# Autodesk Inventor assembly: Робот
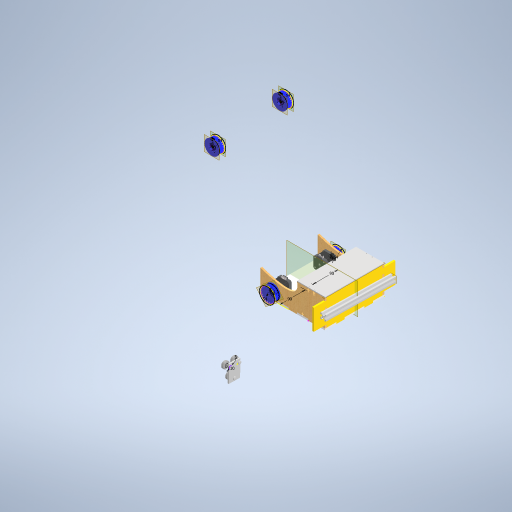
[picture p0: Inventor's stored thumbnail of the model, 512x512]
Saved by Autodesk Inventor 2024.2 (Build 282272000, 272)
## iProperties
Created: 2026-01-27
Part Number: Робот
Document SubType Name: Assembly
Designer: Service
d4: 0,000 мм
Author: Service
## Documents named in this file (9)
- C:\Users\Service\Documents\Artist-v2\3D\Робот.iam
- C:\Users\Service\Documents\Artist-v2\3D\Низ робота.ipt
- C:\Users\Service\Documents\Artist-v2\3D\бок.ipt
- C:\Users\Service\Documents\Artist-v2\3D\перед.ipt
- C:\Users\Service\Documents\Artist-v2\3D\в_профиль 2020.ipt
- C:\Users\Service\Documents\Artist-v2\3D\NEMA17 42-40.ipt
- C:\Users\Service\Documents\Artist-v2\3D\Шестерня.ipt
- C:\Users\Service\Documents\крышка.ipt
- C:\Users\Service\Documents\Artist-v2\3D\каретка.iam
## Components (13 placed, 8 different names)
1. Низ робота:1 — Заподлицо:1, Совмещение:1, Заподлицо:2, Симметрия:1, Совмещение:2, Заподлицо:3, Заподлицо:4, Совмещение:3, Заподлицо:5, Совмещение:12
2. бок:1 — Заподлицо:1, Совмещение:1, Заподлицо:2, Симметрия:1, Совмещение:4, Совмещение:5, Совмещение:13
3. бок:2 — Совмещение:2, Заподлицо:3, Заподлицо:4, Совмещение:6, Совмещение:7, Совмещение:8, Совмещение:10, Заподлицо:6
4. перед:1 — Совмещение:3, Заподлицо:5, Заподлицо:7, Совмещение:18
5. в_профиль 2020:1 — Заподлицо:8, Совмещение:16, Совмещение:17, Совмещение:18
6. NEMA17 42-40:1 — Совмещение:4, Совмещение:5, Совмещение:12, Совмещение:14
7. NEMA17 42-40:2 — Совмещение:6, Совмещение:7, Совмещение:8, Совмещение:9
8. Шестерня:1 — Совмещение:13, Совмещение:14
9. Шестерня:2
10. Шестерня:3
11. Шестерня:4 — Совмещение:9, Совмещение:10
12. крышка:1 — Заподлицо:6, Заподлицо:7
13. каретка:1 [sub-assembly] — Совмещение:15, Касательность:1, Касательность:2
## Relationships (28: Mate 17, Flush 8, Tangent 2, Symmetry 1)
- Заподлицо:1 [Flush]: Низ робота:1 ↔ бок:1
- Совмещение:1 [Mate]: Низ робота:1 ↔ бок:1
- Заподлицо:2 [Flush]: Низ робота:1 ↔ бок:1
- Симметрия:1 [Symmetry]: Низ робота:1 ↔ бок:1
- Совмещение:2 [Mate]: Низ робота:1 ↔ бок:2
- Заподлицо:3 [Flush]: Низ робота:1 ↔ бок:2
- Заподлицо:4 [Flush]: Низ робота:1 ↔ бок:2
- Совмещение:3 [Mate]: Низ робота:1 ↔ перед:1
- Заподлицо:5 [Flush]: Низ робота:1 ↔ перед:1
- Совмещение:4 [Mate]: бок:1 ↔ NEMA17 42-40:1
- Совмещение:5 [Mate]: бок:1 ↔ NEMA17 42-40:1
- Совмещение:6 [Mate]: бок:2 ↔ NEMA17 42-40:2
- Совмещение:7 [Mate]: бок:2 ↔ NEMA17 42-40:2
- Совмещение:8 [Mate]: бок:2 ↔ NEMA17 42-40:2
- Совмещение:9 [Mate]: NEMA17 42-40:2 ↔ Шестерня:4
- Совмещение:10 [Mate]: бок:2 ↔ Шестерня:4
- Совмещение:12 [Mate]: Низ робота:1 ↔ NEMA17 42-40:1
- Совмещение:13 [Mate]: бок:1 ↔ Шестерня:1
- Совмещение:14 [Mate]: NEMA17 42-40:1 ↔ Шестерня:1
- Заподлицо:6 [Flush]: бок:2 ↔ крышка:1
- Заподлицо:7 [Flush]: перед:1 ↔ крышка:1
- Заподлицо:8 [Flush] (-3.9 mm): в_профиль 2020:1
- Совмещение:15 [Mate] (13.2 mm): каретка:1
- Совмещение:16 [Mate]: в_профиль 2020:1
- Совмещение:17 [Mate]: в_профиль 2020:1
- Касательность:1 [Tangent]: каретка:1
- Касательность:2 [Tangent]: каретка:1
- Совмещение:18 [Mate]: перед:1 ↔ в_профиль 2020:1
